# Autodesk Inventor assembly: sprocket and bevel gear on shaft
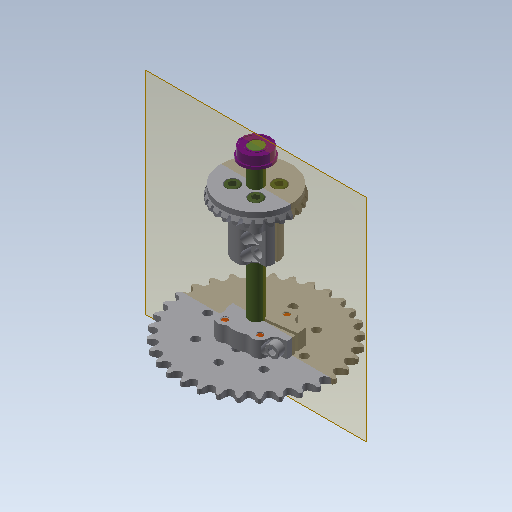
[picture p0: Inventor's stored thumbnail of the model, 512x512]
Saved by Autodesk Inventor 2020 (Build 240168000, 168)
## iProperties
Created: 2019-09-29
Part Number: sprocket and bevel gear on shaft
Document SubType Name: Assembly
Designer: ball
Author: ball
## Documents named in this file (6)
- D:\FTC8863\2019 Robot\Mecanum Drive Train\sprocket and bevel gear on shaft.iam
- D:\FTC8863\2019 Robot\Mecanum Drive Train\bevel gear with clamping hub.iam
- D:\FTC8863\2019 Robot\Mecanum Drive Train\32 spocket with hub.iam
- D:\FTC8863\2019 Robot\Mecanum Drive Train\3_35 shaft.ipt
- D:\FTC8863\Actobotics\535 parts\535198.ipt
- D:\FTC8863\Actobotics\633 parts\633104.ipt
## Components (8 placed, 5 different names)
1. 3_35 shaft:1 — Flush:3, Mate:12, Mate:14, Mate:15, Mate:16, Mate:17, Flush:4
2. bevel gear with clamping hub:1 [sub-assembly] — Flush:5
3. 32 spocket with hub:1 [sub-assembly] — Flush:3, Mate:13
4. 535198:1 — Mate:16
5. 633104:1 — Mate:12, Mate:13
6. 633104:2 — Mate:14
7. 633104:3 — Mate:15
8. 535198:2 — Mate:17, Flush:4, Flush:5
## Relationships (17: Mate 13, Flush 3, Angle 1)
- [Mate]: 3_35 shaft:1 ↔ 32 spocket with hub:1
- [Mate]: 3_35 shaft:1 ↔ bevel gear with clamping hub:1
- [Mate]: 3_35 shaft:1 ↔ bevel gear with clamping hub:1
- [Mate]: 3_35 shaft:1
- [Angle] (90 deg): 3_35 shaft:1
- Flush:3 (9.7028 mm): 3_35 shaft:1 ↔ 32 spocket with hub:1
- [Mate]: 633104:1 ↔ 633104:2
- [Mate]: 633104:2 ↔ 633104:3
- [Mate]: 535198:1 ↔ 633104:3
- Mate:12: 3_35 shaft:1 ↔ 633104:1
- Mate:13: 32 spocket with hub:1 ↔ 633104:1
- Mate:14: 3_35 shaft:1 ↔ 633104:2
- Mate:15: 3_35 shaft:1 ↔ 633104:3
- Mate:16: 3_35 shaft:1 ↔ 535198:1
- Mate:17: 3_35 shaft:1 ↔ 535198:2
- Flush:4: 3_35 shaft:1 ↔ 535198:2
- Flush:5 (11.303 mm): bevel gear with clamping hub:1 ↔ 535198:2
